# Autodesk Inventor assembly: SolarPanel
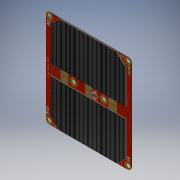
[picture p0: Inventor's stored thumbnail of the model, 180x180]
Saved by Autodesk Inventor 2018 (Build 220112000, 112)
## iProperties
Created: 2018-11-29
Part Number: SolarPanel
Document SubType Name: Assembly
Designer: Bradley
Author: Bradley
## Documents named in this file (21)
- C:\Users\Bradley\Documents\GitHub\CougsInSpace\CougSat1-Hardware\CougSat1-PowerBoard\CADModel\Native\SolarPanel.iam
- C:\Users\Bradley\Documents\GitHub\CougsInSpace\CougSat1-Hardware\CougSat1-PowerBoard\CADModel\Native\SolarPanel_PCB.ipt
- C:\Users\Bradley\Documents\GitHub\CougsInSpace\Resources\ComponentModels\Electronics\SolarCell_UTJ.ipt
- C:\Users\Bradley\Documents\GitHub\CougsInSpace\Resources\ComponentModels\Electronics\Thermistor_1608.ipt
- C:\Users\Bradley\Documents\GitHub\CougsInSpace\Resources\ComponentModels\Electronics\Capacitor_1608-0.8mm.ipt
- C:\Users\Bradley\Documents\GitHub\CougsInSpace\Resources\ComponentModels\Electronics\Resistor_1608-0.5mm.ipt
- C:\Users\Bradley\Documents\GitHub\CougsInSpace\Resources\ComponentModels\Electronics\Photodiode_SFH2430.ipt
- C:\Users\Bradley\Documents\GitHub\CougsInSpace\Resources\ComponentModels\Electronics\Semiconductor_QFN38-5x7.ipt
- C:\Users\Bradley\Documents\GitHub\CougsInSpace\Resources\ComponentModels\Electronics\Semiconductor_WSON-8.ipt
- C:\Users\Bradley\Documents\GitHub\CougsInSpace\Resources\ComponentModels\Electronics\Semiconductor_TSSOP-8.ipt
- C:\Users\Bradley\Documents\GitHub\CougsInSpace\Resources\ComponentModels\Connectors\PicoLock-J-7.ipt
- C:\Users\Bradley\Documents\GitHub\CougsInSpace\Resources\ComponentModels\Connectors\PicoLock-P-7.ipt
- C:\Users\Bradley\Documents\GitHub\CougsInSpace\Resources\ComponentModels\Connectors\PicoLock-J-4.ipt
- C:\Users\Bradley\Documents\GitHub\CougsInSpace\Resources\ComponentModels\Connectors\PicoLock-P-4.ipt
- C:\Users\Bradley\Documents\GitHub\CougsInSpace\Resources\ComponentModels\Electronics\Inductor_6060.ipt
- C:\Users\Bradley\Documents\GitHub\CougsInSpace\Resources\ComponentModels\Electronics\Semiconductor_POWERMITE.ipt
- C:\Users\Bradley\Documents\GitHub\CougsInSpace\Resources\ComponentModels\Electronics\Capacitor_4028-Tantalum.ipt
- C:\Users\Bradley\Documents\GitHub\CougsInSpace\Resources\ComponentModels\Electronics\Resistor_3216-0.65mm.ipt
- C:\Users\Bradley\Documents\GitHub\CougsInSpace\Resources\ComponentModels\Electronics\Capacitor_3216-1.6mm.ipt
- C:\Users\Bradley\Documents\GitHub\CougsInSpace\Resources\ComponentModels\Electronics\Inductor_1608-0.8mm.ipt
- C:\Users\Bradley\Documents\GitHub\CougsInSpace\Resources\ComponentModels\Electronics\ResistorArray-1616.ipt
## Components (104 placed, 20 different names)
1. SolarPanel_PCB:1 — Mate:1, Mate:2, Mate:5, Mate:6, Mate:9, Mate:10, Mate:11, Mate:12, Mate:13, Mate:14, Mate:15, Mate:16, Mate:29, Mate:32, Mate:33, Mate:34, Mate:40, Mate:41, Mate:48, Mate:49, Mate:50, Mate:51, Mate:54, Mate:55, Mate:58, Mate:59, Mate:60, Mate:67, Mate:68, Mate:69, Mate:73, Mate:74, Mate:77, Mate:78, Mate:79, Mate:80, Mate:81, Mate:82, Mate:83, Mate:84, Mate:99, Mate:103, Mate:104, Mate:105, Mate:106, Mate:107, Mate:108, Mate:109, Mate:110, Mate:111, Mate:112, Mate:113, Mate:114, Mate:138, Mate:139, Mate:143, Mate:144, Mate:145, Mate:146, Mate:147, Mate:148, Mate:149, Mate:150, Mate:151, Mate:152, Mate:153, Mate:154, Mate:155, Mate:156, Mate:157, Mate:158, Mate:159, Mate:160, Mate:161, Mate:162, Mate:163, Mate:164, Mate:165, Mate:166, Mate:167, Mate:168, Mate:169, Mate:170, Mate:173, Mate:175, Mate:176, Mate:177, Mate:178, Mate:179, Mate:180, Mate:181, Mate:182, Mate:183, Mate:184, Mate:266, Mate:267, Mate:268, Mate:269, Mate:270, Mate:271, Mate:272
2. PicoLock-J-4:1 — Mate:49, Flush:17, Flush:18
3. PicoLock-J-7:1 — Mate:48, Flush:19, Flush:20
4. PicoLock-P-4:1
5. PicoLock-P-7:1
6. Capacitor_1608-0.8mm:1 — Mate:9, Mate:17, Mate:18
7. Capacitor_1608-0.8mm:2 — Mate:11, Mate:19, Flush:5
8. Capacitor_1608-0.8mm:3 — Mate:13, Flush:6, Mate:20
9. Capacitor_1608-0.8mm:4 — Mate:15, Mate:21, Mate:22
10. Capacitor_1608-0.8mm:6 — Mate:103, Mate:116, Flush:33
11. Capacitor_1608-0.8mm:7 — Mate:104, Mate:117, Mate:118
12. Capacitor_1608-0.8mm:8 — Mate:105, Mate:119, Mate:120
13. Capacitor_1608-0.8mm:9 — Mate:106, Mate:121, Mate:122
14. Capacitor_1608-0.8mm:10 — Mate:107, Mate:123, Flush:34
15. Capacitor_1608-0.8mm:11 — Mate:110, Mate:124, Mate:125
16. Capacitor_1608-0.8mm:12 — Mate:108, Mate:126, Mate:127
17. Capacitor_1608-0.8mm:13 — Mate:109, Mate:128, Flush:35
18. Capacitor_1608-0.8mm:14 — Mate:111, Mate:129, Flush:36
19. Capacitor_1608-0.8mm:15 — Mate:112, Mate:130, Mate:131
20. Capacitor_1608-0.8mm:16 — Mate:113, Mate:132, Mate:133
21. Capacitor_1608-0.8mm:17 — Mate:114, Mate:134, Flush:37
22. Capacitor_3216-1.6mm:1 — Mate:77, Mate:85, Mate:86
23. Capacitor_3216-1.6mm:2 — Mate:78, Mate:87, Flush:30
24. Capacitor_3216-1.6mm:3 — Mate:79, Mate:88, Mate:89
25. Capacitor_3216-1.6mm:4 — Mate:80, Mate:90, Mate:91
26. Capacitor_3216-1.6mm:5 — Mate:81, Mate:92, Mate:93
27. Capacitor_3216-1.6mm:6 — Mate:82, Mate:94, Mate:95
28. Capacitor_3216-1.6mm:7 — Mate:83, Mate:96, Mate:97
29. Capacitor_3216-1.6mm:8 — Mate:84, Mate:98, Flush:31
30. Capacitor_4028-Tantalum:1 — Mate:67, Flush:25, Flush:26
31. Capacitor_4028-Tantalum:2 — Mate:68, Mate:70, Mate:71
32. Capacitor_4028-Tantalum:3 — Mate:69, Flush:27, Mate:72
33. Inductor_1608-0.8mm:1 — Mate:99, Mate:100, Mate:101
34. Inductor_6060:1 — Mate:50, Mate:52, Flush:21
35. Inductor_6060:2 — Mate:51, Mate:53, Flush:22
36. Photodiode_SFH2430:1 — Mate:29, Mate:30, Flush:9
37. Resistor_1608-0.5mm:1 — Mate:10, Mate:23, Flush:7
38. Resistor_1608-0.5mm:2 — Mate:12, Mate:24, Mate:25
39. Resistor_1608-0.5mm:3 — Mate:14, Mate:26, Mate:27
40. Resistor_1608-0.5mm:4 — Mate:16, Mate:28, Flush:8
41. Resistor_1608-0.5mm:7 — Mate:139, Mate:189, Mate:190
42. Resistor_1608-0.5mm:10 — Mate:138, Mate:193, Mate:194
43. Resistor_1608-0.5mm:13 — Mate:143, Mate:197, Flush:42
44. Resistor_1608-0.5mm:14 — Mate:144, Mate:198, Flush:43
45. Resistor_1608-0.5mm:15 — Mate:145, Mate:199, Flush:44
46. Resistor_1608-0.5mm:16 — Mate:149, Mate:200, Mate:201
47. Resistor_1608-0.5mm:17 — Mate:150, Mate:202, Mate:203
48. Resistor_1608-0.5mm:18 — Mate:151, Mate:204, Mate:205
49. Resistor_1608-0.5mm:19 — Mate:146, Mate:206, Flush:45
50. Resistor_1608-0.5mm:20 — Mate:147, Mate:207, Mate:208
51. Resistor_1608-0.5mm:21 — Mate:148, Mate:209, Mate:210
52. Resistor_1608-0.5mm:22 — Mate:155, Mate:211, Flush:46
53. Resistor_1608-0.5mm:23 — Mate:156, Mate:212, Mate:213
54. Resistor_1608-0.5mm:24 — Mate:152, Mate:214, Mate:215
55. Resistor_1608-0.5mm:25 — Mate:157, Mate:216, Flush:47
56. Resistor_1608-0.5mm:26 — Mate:158, Mate:217, Flush:48
57. Resistor_1608-0.5mm:27 — Mate:163, Mate:218, Flush:49
58. Resistor_1608-0.5mm:28 — Mate:161, Mate:219, Mate:220
59. Resistor_1608-0.5mm:29 — Mate:162, Mate:221, Mate:222
60. Resistor_1608-0.5mm:30 — Mate:164, Mate:223, Mate:224
61. Resistor_1608-0.5mm:31 — Mate:165, Mate:225, Mate:226
62. Resistor_1608-0.5mm:32 — Mate:160, Mate:227, Flush:50
63. Resistor_1608-0.5mm:33 — Mate:159, Mate:228, Flush:51
64. Resistor_1608-0.5mm:34 — Mate:154, Mate:229, Mate:230
65. Resistor_1608-0.5mm:35 — Mate:153, Mate:231, Mate:232
66. Resistor_1608-0.5mm:36 — Mate:169, Mate:233, Flush:52
67. Resistor_1608-0.5mm:37 — Mate:170, Mate:234, Flush:53
68. Resistor_1608-0.5mm:40 — Mate:175, Mate:238, Flush:55
69. Resistor_1608-0.5mm:41 — Mate:173, Mate:239, Mate:240
70. Resistor_1608-0.5mm:43 — Mate:179, Mate:242, Mate:243
71. Resistor_1608-0.5mm:44 — Mate:180, Mate:244, Mate:245
72. Resistor_1608-0.5mm:45 — Mate:184, Mate:246, Mate:247
73. Resistor_1608-0.5mm:46 — Mate:183, Mate:248, Mate:249
74. Resistor_1608-0.5mm:47 — Mate:182, Mate:250, Mate:251
75. Resistor_1608-0.5mm:48 — Mate:181, Mate:252, Mate:253
76. Resistor_1608-0.5mm:49 — Mate:176, Mate:254, Mate:255
77. Resistor_1608-0.5mm:50 — Mate:177, Mate:256, Mate:257
78. Resistor_1608-0.5mm:51 — Mate:178, Mate:258, Mate:259
79. Resistor_1608-0.5mm:52 — Mate:168, Mate:260, Mate:261
80. Resistor_1608-0.5mm:53 — Mate:167, Mate:262, Mate:263
81. Resistor_1608-0.5mm:54 — Mate:166, Mate:264, Mate:265
82. Resistor_3216-0.65mm:1 — Mate:73, Mate:75, Flush:28
83. Resistor_3216-0.65mm:2 — Mate:74, Mate:76, Flush:29
84. ResistorArray-1616:1 — Mate:266, Mate:273, Mate:274
85. ResistorArray-1616:2 — Mate:267, Mate:275, Mate:276
86. ResistorArray-1616:3 — Mate:268, Mate:277, Flush:56
87. ResistorArray-1616:4 — Mate:269, Mate:278, Mate:279
88. ResistorArray-1616:5 — Mate:270, Mate:280, Flush:57
89. ResistorArray-1616:6 — Mate:271, Mate:281, Mate:282
90. ResistorArray-1616:7 — Mate:272, Mate:283, Flush:58
91. Semiconductor_POWERMITE:1 — Mate:54, Mate:56, Mate:57
92. Semiconductor_POWERMITE:2 — Mate:55, Flush:23, Flush:24
93. Semiconductor_QFN38-5x7:1 — Mate:32, Mate:36, Flush:11
94. Semiconductor_QFN38-5x7:2 — Mate:33, Mate:37, Flush:12
95. Semiconductor_TSSOP-8:1 — Mate:40, Mate:42, Flush:13
96. Semiconductor_TSSOP-8:2 — Mate:41, Flush:14, Mate:43
97. Semiconductor_WSON-8:1 — Mate:34, Mate:38, Mate:39
98. SolarCell_UTJ:1 — Mate:1, Mate:3, Mate:4
99. SolarCell_UTJ:2 — Mate:2, Flush:1, Flush:2
100. Thermistor_1608:1 — Mate:6, Mate:7, Flush:3
101. Thermistor_1608:2 — Mate:5, Mate:8, Flush:4
102. Thermistor_1608:3 — Mate:58, Mate:61, Mate:62
103. Thermistor_1608:4 — Mate:59, Mate:63, Mate:64
104. Thermistor_1608:5 — Mate:60, Mate:65, Mate:66
## Relationships (309: Mate 258, Flush 51)
- Mate:1: SolarPanel_PCB:1 ↔ SolarCell_UTJ:1
- Mate:2: SolarPanel_PCB:1 ↔ SolarCell_UTJ:2
- Mate:3: SolarCell_UTJ:1
- Flush:1: SolarCell_UTJ:2
- Flush:2 (5 mm): SolarCell_UTJ:2
- Mate:4 (5 mm): SolarCell_UTJ:1
- Mate:5: SolarPanel_PCB:1 ↔ Thermistor_1608:2
- Mate:6: SolarPanel_PCB:1 ↔ Thermistor_1608:1
- Mate:7 (31 mm): Thermistor_1608:1
- Flush:3 (-43.5 mm): Thermistor_1608:1
- Mate:8 (-31.125 mm): Thermistor_1608:2
- Flush:4 (43.8 mm): Thermistor_1608:2
- Mate:9: SolarPanel_PCB:1 ↔ Capacitor_1608-0.8mm:1
- Mate:10: SolarPanel_PCB:1 ↔ Resistor_1608-0.5mm:1
- Mate:11: SolarPanel_PCB:1 ↔ Capacitor_1608-0.8mm:2
- Mate:12: SolarPanel_PCB:1 ↔ Resistor_1608-0.5mm:2
- Mate:13: SolarPanel_PCB:1 ↔ Capacitor_1608-0.8mm:3
- Mate:14: SolarPanel_PCB:1 ↔ Resistor_1608-0.5mm:3
- Mate:15: SolarPanel_PCB:1 ↔ Capacitor_1608-0.8mm:4
- Mate:16: SolarPanel_PCB:1 ↔ Resistor_1608-0.5mm:4
- Mate:17 (38.15 mm): Capacitor_1608-0.8mm:1
- Mate:18 (36.7 mm): Capacitor_1608-0.8mm:1
- Mate:19 (-37 mm): Capacitor_1608-0.8mm:2
- Flush:5 (-35.25 mm): Capacitor_1608-0.8mm:2
- Flush:6 (-37 mm): Capacitor_1608-0.8mm:3
- Mate:20 (-35.25 mm): Capacitor_1608-0.8mm:3
- Mate:21 (-36.7 mm): Capacitor_1608-0.8mm:4
- Mate:22 (-38.2 mm): Capacitor_1608-0.8mm:4
- Mate:23 (-37 mm): Resistor_1608-0.5mm:1
- Flush:7 (37.25 mm): Resistor_1608-0.5mm:1
- Mate:24 (33.05 mm): Resistor_1608-0.5mm:2
- Mate:25 (38.15 mm): Resistor_1608-0.5mm:2
- Mate:26 (-33 mm): Resistor_1608-0.5mm:3
- Mate:27 (-38.2 mm): Resistor_1608-0.5mm:3
- Mate:28 (37 mm): Resistor_1608-0.5mm:4
- Flush:8 (37.25 mm): Resistor_1608-0.5mm:4
- Mate:29: SolarPanel_PCB:1 ↔ Photodiode_SFH2430:1
- Mate:30 (-0.25 mm): Photodiode_SFH2430:1
- Flush:9 (-6.25 mm): Photodiode_SFH2430:1
- Mate:32: SolarPanel_PCB:1 ↔ Semiconductor_QFN38-5x7:1
- Mate:33: SolarPanel_PCB:1 ↔ Semiconductor_QFN38-5x7:2
- Mate:34: SolarPanel_PCB:1 ↔ Semiconductor_WSON-8:1
- Mate:36 (26 mm): Semiconductor_QFN38-5x7:1
- Flush:11 (-19 mm): Semiconductor_QFN38-5x7:1
- Mate:37 (27 mm): Semiconductor_QFN38-5x7:2
- Flush:12 (-9 mm): Semiconductor_QFN38-5x7:2
- Mate:38 (5.25 mm): Semiconductor_WSON-8:1
- Mate:39 (29.5 mm): Semiconductor_WSON-8:1
- Mate:40: SolarPanel_PCB:1 ↔ Semiconductor_TSSOP-8:1
- Mate:41: SolarPanel_PCB:1 ↔ Semiconductor_TSSOP-8:2
- Mate:42 (-10 mm): Semiconductor_TSSOP-8:1
- Flush:13 (10.5 mm): Semiconductor_TSSOP-8:1
- Flush:14 (-10 mm): Semiconductor_TSSOP-8:2
- Mate:43 (10.5 mm): Semiconductor_TSSOP-8:2
- [Flush]: PicoLock-J-7:1 ↔ PicoLock-P-7:1
- [Mate]: PicoLock-J-7:1 ↔ PicoLock-P-7:1
- [Mate] (0.025 mm): PicoLock-J-7:1 ↔ PicoLock-P-7:1
- [Flush]: PicoLock-J-4:1 ↔ PicoLock-P-4:1
- [Mate]: PicoLock-J-4:1 ↔ PicoLock-P-4:1
- [Mate] (0.025 mm): PicoLock-J-4:1 ↔ PicoLock-P-4:1
- Mate:48: SolarPanel_PCB:1 ↔ PicoLock-J-7:1
- Mate:49: SolarPanel_PCB:1 ↔ PicoLock-J-4:1
- Flush:17 (26 mm): PicoLock-J-4:1
- Flush:18 (-1 mm): PicoLock-J-4:1
- Flush:19 (11.75 mm): PicoLock-J-7:1
- Flush:20 (-1 mm): PicoLock-J-7:1
- Mate:50: SolarPanel_PCB:1 ↔ Inductor_6060:1
- Mate:51: SolarPanel_PCB:1 ↔ Inductor_6060:2
- Mate:52 (-16.25 mm): Inductor_6060:1
- Flush:21 (8 mm): Inductor_6060:1
- Mate:53 (16.25 mm): Inductor_6060:2
- Flush:22 (-8 mm): Inductor_6060:2
- Mate:54: SolarPanel_PCB:1 ↔ Semiconductor_POWERMITE:1
- Mate:55: SolarPanel_PCB:1 ↔ Semiconductor_POWERMITE:2
- Mate:56 (-2.75 mm): Semiconductor_POWERMITE:1
- Mate:57 (-1.5 mm): Semiconductor_POWERMITE:1
- Flush:23 (-3.25 mm): Semiconductor_POWERMITE:2
- Flush:24 (1.5 mm): Semiconductor_POWERMITE:2
- Mate:58: SolarPanel_PCB:1 ↔ Thermistor_1608:3
- Mate:59: SolarPanel_PCB:1 ↔ Thermistor_1608:4
- Mate:60: SolarPanel_PCB:1 ↔ Thermistor_1608:5
- Mate:61 (-10.75 mm): Thermistor_1608:3
- Mate:62 (-4.75 mm): Thermistor_1608:3
- Mate:63 (1.85 mm): Thermistor_1608:4
- Mate:64 (-2.6 mm): Thermistor_1608:4
- Mate:65 (10.75 mm): Thermistor_1608:5
- Mate:66 (4.75 mm): Thermistor_1608:5
- Mate:67: SolarPanel_PCB:1 ↔ Capacitor_4028-Tantalum:1
- Mate:68: SolarPanel_PCB:1 ↔ Capacitor_4028-Tantalum:2
- Mate:69: SolarPanel_PCB:1 ↔ Capacitor_4028-Tantalum:3
- Flush:25 (6.75 mm): Capacitor_4028-Tantalum:1
- Flush:26 (27 mm): Capacitor_4028-Tantalum:1
- Mate:70 (6.75 mm): Capacitor_4028-Tantalum:2
- Mate:71 (27 mm): Capacitor_4028-Tantalum:2
- Flush:27 (16.25 mm): Capacitor_4028-Tantalum:3
- Mate:72 (22.75 mm): Capacitor_4028-Tantalum:3
- Mate:73: SolarPanel_PCB:1 ↔ Resistor_3216-0.65mm:1
- Mate:74: SolarPanel_PCB:1 ↔ Resistor_3216-0.65mm:2
- Mate:75 (-8.5 mm): Resistor_3216-0.65mm:1
- Flush:28 (7 mm): Resistor_3216-0.65mm:1
- Mate:76 (8.5 mm): Resistor_3216-0.65mm:2
- Flush:29 (-7 mm): Resistor_3216-0.65mm:2
- Mate:77: SolarPanel_PCB:1 ↔ Capacitor_3216-1.6mm:1
- Mate:78: SolarPanel_PCB:1 ↔ Capacitor_3216-1.6mm:2
- Mate:79: SolarPanel_PCB:1 ↔ Capacitor_3216-1.6mm:3
- Mate:80: SolarPanel_PCB:1 ↔ Capacitor_3216-1.6mm:4
- Mate:81: SolarPanel_PCB:1 ↔ Capacitor_3216-1.6mm:5
- Mate:82: SolarPanel_PCB:1 ↔ Capacitor_3216-1.6mm:6
- Mate:83: SolarPanel_PCB:1 ↔ Capacitor_3216-1.6mm:7
- Mate:84: SolarPanel_PCB:1 ↔ Capacitor_3216-1.6mm:8
- Mate:85 (24.5 mm): Capacitor_3216-1.6mm:1
- Mate:86 (-7 mm): Capacitor_3216-1.6mm:1
- Mate:87 (-6.75 mm): Capacitor_3216-1.6mm:2
- Flush:30 (23.5 mm): Capacitor_3216-1.6mm:2
- Mate:88 (-5.75 mm): Capacitor_3216-1.6mm:3
- Mate:89 (-4.25 mm): Capacitor_3216-1.6mm:3
- Mate:90 (-5.75 mm): Capacitor_3216-1.6mm:4
- Mate:91 (-1.25 mm): Capacitor_3216-1.6mm:4
- Mate:92 (-5.75 mm): Capacitor_3216-1.6mm:5
- Mate:93 (1.75 mm): Capacitor_3216-1.6mm:5
- Mate:94 (-5.75 mm): Capacitor_3216-1.6mm:6
- Mate:95 (4.75 mm): Capacitor_3216-1.6mm:6
- Mate:96 (-19.75 mm): Capacitor_3216-1.6mm:7
- Mate:97 (5.75 mm): Capacitor_3216-1.6mm:7
- Mate:98 (6.75 mm): Capacitor_3216-1.6mm:8
- Flush:31 (-23.5 mm): Capacitor_3216-1.6mm:8
- Mate:99: SolarPanel_PCB:1 ↔ Inductor_1608-0.8mm:1
- Mate:100 (-13.5 mm): Inductor_1608-0.8mm:1
- Mate:101 (16.25 mm): Inductor_1608-0.8mm:1
- Mate:103: SolarPanel_PCB:1 ↔ Capacitor_1608-0.8mm:6
- Mate:104: SolarPanel_PCB:1 ↔ Capacitor_1608-0.8mm:7
- Mate:105: SolarPanel_PCB:1 ↔ Capacitor_1608-0.8mm:8
- Mate:106: SolarPanel_PCB:1 ↔ Capacitor_1608-0.8mm:9
- Mate:107: SolarPanel_PCB:1 ↔ Capacitor_1608-0.8mm:10
- Mate:108: SolarPanel_PCB:1 ↔ Capacitor_1608-0.8mm:12
- Mate:109: SolarPanel_PCB:1 ↔ Capacitor_1608-0.8mm:13
- Mate:110: SolarPanel_PCB:1 ↔ Capacitor_1608-0.8mm:11
- Mate:111: SolarPanel_PCB:1 ↔ Capacitor_1608-0.8mm:14
- Mate:112: SolarPanel_PCB:1 ↔ Capacitor_1608-0.8mm:15
- Mate:113: SolarPanel_PCB:1 ↔ Capacitor_1608-0.8mm:16
- Mate:114: SolarPanel_PCB:1 ↔ Capacitor_1608-0.8mm:17
- Mate:116 (-19 mm): Capacitor_1608-0.8mm:6
- Flush:33 (7.25 mm): Capacitor_1608-0.8mm:6
- Mate:117 (-19.5 mm): Capacitor_1608-0.8mm:7
- Mate:118 (-16.5 mm): Capacitor_1608-0.8mm:7
- Mate:119 (-10.5 mm): Capacitor_1608-0.8mm:8
- Mate:120 (-15.25 mm): Capacitor_1608-0.8mm:8
- Mate:121 (17 mm): Capacitor_1608-0.8mm:9
- Mate:122 (-5.25 mm): Capacitor_1608-0.8mm:9
- Mate:123 (6.25 mm): Capacitor_1608-0.8mm:10
- Flush:34 (16 mm): Capacitor_1608-0.8mm:10
- Mate:124 (10.5 mm): Capacitor_1608-0.8mm:11
- Mate:125 (15.25 mm): Capacitor_1608-0.8mm:11
- Mate:126 (15.5 mm): Capacitor_1608-0.8mm:12
- Mate:127 (18 mm): Capacitor_1608-0.8mm:12
- Mate:128 (19 mm): Capacitor_1608-0.8mm:13
- Flush:35 (-7.25 mm): Capacitor_1608-0.8mm:13
- Mate:129 (19 mm): Capacitor_1608-0.8mm:14
- Flush:36 (15.25 mm): Capacitor_1608-0.8mm:14
- Mate:130 (19 mm): Capacitor_1608-0.8mm:15
- Mate:131 (21.75 mm): Capacitor_1608-0.8mm:15
- Mate:132 (-11.75 mm): Capacitor_1608-0.8mm:16
- Mate:133 (22.75 mm): Capacitor_1608-0.8mm:16
- Mate:134 (26 mm): Capacitor_1608-0.8mm:17
- Flush:37 (-6 mm): Capacitor_1608-0.8mm:17
- Mate:138: SolarPanel_PCB:1 ↔ Resistor_1608-0.5mm:10
- Mate:139: SolarPanel_PCB:1 ↔ Resistor_1608-0.5mm:7
- Mate:143: SolarPanel_PCB:1 ↔ Resistor_1608-0.5mm:13
- Mate:144: SolarPanel_PCB:1 ↔ Resistor_1608-0.5mm:14
- Mate:145: SolarPanel_PCB:1 ↔ Resistor_1608-0.5mm:15
- Mate:146: SolarPanel_PCB:1 ↔ Resistor_1608-0.5mm:19
- Mate:147: SolarPanel_PCB:1 ↔ Resistor_1608-0.5mm:20
- Mate:148: SolarPanel_PCB:1 ↔ Resistor_1608-0.5mm:21
- Mate:149: SolarPanel_PCB:1 ↔ Resistor_1608-0.5mm:16
- Mate:150: SolarPanel_PCB:1 ↔ Resistor_1608-0.5mm:17
- Mate:151: SolarPanel_PCB:1 ↔ Resistor_1608-0.5mm:18
- Mate:152: SolarPanel_PCB:1 ↔ Resistor_1608-0.5mm:24
- Mate:153: SolarPanel_PCB:1 ↔ Resistor_1608-0.5mm:35
- Mate:154: SolarPanel_PCB:1 ↔ Resistor_1608-0.5mm:34
- Mate:155: SolarPanel_PCB:1 ↔ Resistor_1608-0.5mm:22
- Mate:156: SolarPanel_PCB:1 ↔ Resistor_1608-0.5mm:23
- Mate:157: SolarPanel_PCB:1 ↔ Resistor_1608-0.5mm:25
- Mate:158: SolarPanel_PCB:1 ↔ Resistor_1608-0.5mm:26
- Mate:159: SolarPanel_PCB:1 ↔ Resistor_1608-0.5mm:33
- Mate:160: SolarPanel_PCB:1 ↔ Resistor_1608-0.5mm:32
- Mate:161: SolarPanel_PCB:1 ↔ Resistor_1608-0.5mm:28
- Mate:162: SolarPanel_PCB:1 ↔ Resistor_1608-0.5mm:29
- Mate:163: SolarPanel_PCB:1 ↔ Resistor_1608-0.5mm:27
- Mate:164: SolarPanel_PCB:1 ↔ Resistor_1608-0.5mm:30
- Mate:165: SolarPanel_PCB:1 ↔ Resistor_1608-0.5mm:31
- Mate:166: SolarPanel_PCB:1 ↔ Resistor_1608-0.5mm:54
- Mate:167: SolarPanel_PCB:1 ↔ Resistor_1608-0.5mm:53
- Mate:168: SolarPanel_PCB:1 ↔ Resistor_1608-0.5mm:52
- Mate:169: SolarPanel_PCB:1 ↔ Resistor_1608-0.5mm:36
- Mate:170: SolarPanel_PCB:1 ↔ Resistor_1608-0.5mm:37
- Mate:173: SolarPanel_PCB:1 ↔ Resistor_1608-0.5mm:41
- Mate:175: SolarPanel_PCB:1 ↔ Resistor_1608-0.5mm:40
- Mate:176: SolarPanel_PCB:1 ↔ Resistor_1608-0.5mm:49
- Mate:177: SolarPanel_PCB:1 ↔ Resistor_1608-0.5mm:50
- Mate:178: SolarPanel_PCB:1 ↔ Resistor_1608-0.5mm:51
- Mate:179: SolarPanel_PCB:1 ↔ Resistor_1608-0.5mm:43
- Mate:180: SolarPanel_PCB:1 ↔ Resistor_1608-0.5mm:44
- Mate:181: SolarPanel_PCB:1 ↔ Resistor_1608-0.5mm:48
- Mate:182: SolarPanel_PCB:1 ↔ Resistor_1608-0.5mm:47
- Mate:183: SolarPanel_PCB:1 ↔ Resistor_1608-0.5mm:46
- Mate:184: SolarPanel_PCB:1 ↔ Resistor_1608-0.5mm:45
- Mate:189 (-1.75 mm): Resistor_1608-0.5mm:7
- Mate:190 (-24.9 mm): Resistor_1608-0.5mm:7
- Mate:193 (-1.75 mm): Resistor_1608-0.5mm:10
- Mate:194 (-22.9 mm): Resistor_1608-0.5mm:10
- Mate:197 (-19 mm): Resistor_1608-0.5mm:13
- Flush:42 (5.25 mm): Resistor_1608-0.5mm:13
- Mate:198 (-18 mm): Resistor_1608-0.5mm:14
- Flush:43 (9.5 mm): Resistor_1608-0.5mm:14
- Mate:199 (-18 mm): Resistor_1608-0.5mm:15
- Flush:44 (11.5 mm): Resistor_1608-0.5mm:15
- Mate:200 (-6.5 mm): Resistor_1608-0.5mm:16
- Mate:201 (-16.25 mm): Resistor_1608-0.5mm:16
- Mate:202 (-21.5 mm): Resistor_1608-0.5mm:17
- Mate:203 (-14.5 mm): Resistor_1608-0.5mm:17
- Mate:204 (-6.5 mm): Resistor_1608-0.5mm:18
- Mate:205 (-14.25 mm): Resistor_1608-0.5mm:18
- Mate:206 (-13.75 mm): Resistor_1608-0.5mm:19
- Flush:45 (18.75 mm): Resistor_1608-0.5mm:19
- Mate:207 (-6.5 mm): Resistor_1608-0.5mm:20
- Mate:208 (-12.25 mm): Resistor_1608-0.5mm:20
- Mate:209 (-1.75 mm): Resistor_1608-0.5mm:21
- Mate:210 (-10.75 mm): Resistor_1608-0.5mm:21
- Mate:211 (-9.25 mm): Resistor_1608-0.5mm:22
- Flush:46 (21 mm): Resistor_1608-0.5mm:22
- Mate:212 (-1.75 mm): Resistor_1608-0.5mm:23
- Mate:213 (-8.75 mm): Resistor_1608-0.5mm:23
- Mate:214 (13.25 mm): Resistor_1608-0.5mm:24
- Mate:215 (-5.25 mm): Resistor_1608-0.5mm:24
- Mate:216 (0.25 mm): Resistor_1608-0.5mm:25
- Flush:47 (-8.75 mm): Resistor_1608-0.5mm:25
- Mate:217 (6.25 mm): Resistor_1608-0.5mm:26
- Flush:48 (14 mm): Resistor_1608-0.5mm:26
- Mate:218 (9.25 mm): Resistor_1608-0.5mm:27
- Flush:49 (-21 mm): Resistor_1608-0.5mm:27
- Mate:219 (-16.5 mm): Resistor_1608-0.5mm:28
- Mate:220 (11.75 mm): Resistor_1608-0.5mm:28
- Mate:221 (6.5 mm): Resistor_1608-0.5mm:29
- Mate:222 (12.25 mm): Resistor_1608-0.5mm:29
- Mate:223 (-17.5 mm): Resistor_1608-0.5mm:30
- Mate:224 (13.75 mm): Resistor_1608-0.5mm:30
- Mate:225 (6.5 mm): Resistor_1608-0.5mm:31
- Mate:226 (14.25 mm): Resistor_1608-0.5mm:31
- Mate:227 (15.25 mm): Resistor_1608-0.5mm:32
- Flush:50 (-16.5 mm): Resistor_1608-0.5mm:32
- Mate:228 (15.25 mm): Resistor_1608-0.5mm:33
- Flush:51 (-14.5 mm): Resistor_1608-0.5mm:33
- Mate:229 (-17.5 mm): Resistor_1608-0.5mm:34
- Mate:230 (15.75 mm): Resistor_1608-0.5mm:34
- Mate:231 (6.5 mm): Resistor_1608-0.5mm:35
- Mate:232 (16.25 mm): Resistor_1608-0.5mm:35
- Mate:233 (18 mm): Resistor_1608-0.5mm:36
- Flush:52 (-11.5 mm): Resistor_1608-0.5mm:36
- Mate:234 (18 mm): Resistor_1608-0.5mm:37
- Flush:53 (-9.5 mm): Resistor_1608-0.5mm:37
- Mate:238 (19 mm): Resistor_1608-0.5mm:40
- Flush:55 (-5.25 mm): Resistor_1608-0.5mm:40
- Mate:239 (-8.6 mm): Resistor_1608-0.5mm:41
- Mate:240 (20.8 mm): Resistor_1608-0.5mm:41
- Mate:242 (12.75 mm): Resistor_1608-0.5mm:43
- Mate:243 (25.25 mm): Resistor_1608-0.5mm:43
- Mate:244 (9 mm): Resistor_1608-0.5mm:44
- Mate:245 (25.25 mm): Resistor_1608-0.5mm:44
- Mate:246 (-15 mm): Resistor_1608-0.5mm:45
- Mate:247 (26.25 mm): Resistor_1608-0.5mm:45
- Mate:248 (-18.75 mm): Resistor_1608-0.5mm:46
- Mate:249 (26.25 mm): Resistor_1608-0.5mm:46
- Mate:250 (12.75 mm): Resistor_1608-0.5mm:47
- Mate:251 (27.75 mm): Resistor_1608-0.5mm:47
- Mate:252 (9 mm): Resistor_1608-0.5mm:48
- Mate:253 (27.75 mm): Resistor_1608-0.5mm:48
- Mate:254 (-15 mm): Resistor_1608-0.5mm:49
- Mate:255 (28.75 mm): Resistor_1608-0.5mm:49
- Mate:256 (-18.75 mm): Resistor_1608-0.5mm:50
- Mate:257 (28.75 mm): Resistor_1608-0.5mm:50
- Mate:258 (12.75 mm): Resistor_1608-0.5mm:51
- Mate:259 (29.75 mm): Resistor_1608-0.5mm:51
- Mate:260 (9 mm): Resistor_1608-0.5mm:52
- Mate:261 (29.75 mm): Resistor_1608-0.5mm:52
- Mate:262 (-15 mm): Resistor_1608-0.5mm:53
- Mate:263 (30.75 mm): Resistor_1608-0.5mm:53
- Mate:264 (-18.75 mm): Resistor_1608-0.5mm:54
- Mate:265 (30.75 mm): Resistor_1608-0.5mm:54
- Mate:266: SolarPanel_PCB:1 ↔ ResistorArray-1616:1
- Mate:267: SolarPanel_PCB:1 ↔ ResistorArray-1616:2
- Mate:268: SolarPanel_PCB:1 ↔ ResistorArray-1616:3
- Mate:269: SolarPanel_PCB:1 ↔ ResistorArray-1616:4
- Mate:270: SolarPanel_PCB:1 ↔ ResistorArray-1616:5
- Mate:271: SolarPanel_PCB:1 ↔ ResistorArray-1616:6
- Mate:272: SolarPanel_PCB:1 ↔ ResistorArray-1616:7
- Mate:273 (18.3 mm): ResistorArray-1616:1
- Mate:274 (-7.2 mm): ResistorArray-1616:1
- Mate:275 (18.3 mm): ResistorArray-1616:2
- Mate:276 (-10.2 mm): ResistorArray-1616:2
- Mate:277 (18.2 mm): ResistorArray-1616:3
- Flush:56 (1.5 mm): ResistorArray-1616:3
- Mate:278 (22.9 mm): ResistorArray-1616:4
- Mate:279 (-0.6 mm): ResistorArray-1616:4
- Mate:280 (-22.2 mm): ResistorArray-1616:5
- Flush:57 (-25.6 mm): ResistorArray-1616:5
- Mate:281 (28.3 mm): ResistorArray-1616:6
- Mate:282 (-1.9 mm): ResistorArray-1616:6
- Mate:283 (-22.9 mm): ResistorArray-1616:7
- Flush:58 (-28.8 mm): ResistorArray-1616:7
## Named parameters: d15_d12 = 0 mm, d16_d13 = 0 mm, d17_d14 = 0.025 mm, d60_d9 = 0 mm, d61_d10 = 0 mm, d62_d11 = 0.025 mm
